# Autodesk Inventor assembly: R-wing
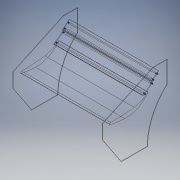
[picture p0: Inventor's stored thumbnail of the model, 180x180]
Saved by Autodesk Inventor 2018.1 (Build 221171000, 171)
## iProperties
Created: 2017-11-02
Part Number: R-wing
Material: 一般
Document SubType Name: Assembly
Designer: kuwano
Author: kuwano
## Documents named in this file (7)
- D:\ku_sk\ドキュメント\Inventor\AeroCAD2018\CAD\Inventor\Aero Parts\R-wing\type6\R-wing.iam
- D:\ku_sk\ドキュメント\Inventor\AeroCAD2018\CAD\Inventor\Aero Parts\R-wing\type6\parts\element_r_1.ipt
- D:\ku_sk\ドキュメント\Inventor\AeroCAD2018\CAD\Inventor\Aero Parts\R-wing\type6\parts\element_r_2.ipt
- D:\ku_sk\ドキュメント\Inventor\AeroCAD2018\CAD\Inventor\Aero Parts\R-wing\type6\parts\end_plate.ipt
- D:\ku_sk\ドキュメント\Inventor\AeroCAD2018\CAD\Inventor\Aero Parts\R-wing\type6\parts\end_plate_MIR.ipt
- D:\ku_sk\ドキュメント\Inventor\AeroCAD2018\CAD\Inventor\Aero Parts\R-wing\type6\parts\cover_re.ipt
- D:\ku_sk\ドキュメント\Inventor\AeroCAD2018\CAD\Inventor\Aero Parts\R-wing\type6\parts\element_clip.ipt
## Components (13 placed, 6 different names)
1. element_r_1:1 — フラッシュ:1, メイト:1, メイト:2, メイト:6, メイト:8, メイト:12, メイト:16, メイト:22, メイト:24, メイト:28, メイト:30
2. element_r_2:1 — フラッシュ:2, メイト:3, メイト:5, メイト:11, メイト:15, メイト:19, メイト:21, メイト:25, メイト:27
3. end_plate:1 — フラッシュ:3, フラッシュ:4, メイト:2, フラッシュ:6, メイト:13, メイト:14, メイト:17, メイト:18, メイト:26, メイト:29
4. end_plate_MIR:1 — フラッシュ:3, フラッシュ:4, メイト:1, メイト:4, メイト:7, メイト:9, メイト:10, メイト:20, メイト:23
5. cover_re:1 — フラッシュ:5
6. element_clip:1 — メイト:3, メイト:4, メイト:5, メイト:10
7. element_clip:2 — メイト:6, メイト:7, メイト:8, メイト:9
8. element_clip:3 — メイト:11, メイト:14, メイト:15, メイト:18
9. element_clip:4 — メイト:12, メイト:13, メイト:16, メイト:17
10. element_clip:5 — メイト:19, メイト:20, メイト:21
11. element_clip:6 — メイト:22, メイト:23, メイト:24
12. element_clip:7 — メイト:25, メイト:26, メイト:27
13. element_clip:8 — メイト:28, メイト:29, メイト:30
## Relationships (36: Mate 30, Flush 6)
- フラッシュ:1 [Flush]: element_r_1:1
- フラッシュ:2 [Flush]: element_r_2:1
- フラッシュ:3 [Flush]: end_plate:1 ↔ end_plate_MIR:1
- フラッシュ:4 [Flush]: end_plate:1 ↔ end_plate_MIR:1
- メイト:1 [Mate]: element_r_1:1 ↔ end_plate_MIR:1
- メイト:2 [Mate]: element_r_1:1 ↔ end_plate:1
- フラッシュ:5 [Flush]: cover_re:1
- メイト:3 [Mate]: element_r_2:1 ↔ element_clip:1
- メイト:4 [Mate]: end_plate_MIR:1 ↔ element_clip:1
- メイト:5 [Mate]: element_r_2:1 ↔ element_clip:1
- メイト:6 [Mate]: element_r_1:1 ↔ element_clip:2
- メイト:7 [Mate]: end_plate_MIR:1 ↔ element_clip:2
- メイト:8 [Mate]: element_r_1:1 ↔ element_clip:2
- メイト:9 [Mate]: end_plate_MIR:1 ↔ element_clip:2
- メイト:10 [Mate]: end_plate_MIR:1 ↔ element_clip:1
- フラッシュ:6 [Flush]: end_plate:1
- メイト:11 [Mate]: element_r_2:1 ↔ element_clip:3
- メイト:12 [Mate]: element_r_1:1 ↔ element_clip:4
- メイト:13 [Mate]: end_plate:1 ↔ element_clip:4
- メイト:14 [Mate]: end_plate:1 ↔ element_clip:3
- メイト:15 [Mate]: element_r_2:1 ↔ element_clip:3
- メイト:16 [Mate]: element_r_1:1 ↔ element_clip:4
- メイト:17 [Mate]: end_plate:1 ↔ element_clip:4
- メイト:18 [Mate]: end_plate:1 ↔ element_clip:3
- メイト:19 [Mate]: element_r_2:1 ↔ element_clip:5
- メイト:20 [Mate]: end_plate_MIR:1 ↔ element_clip:5
- メイト:21 [Mate]: element_r_2:1 ↔ element_clip:5
- メイト:22 [Mate]: element_r_1:1 ↔ element_clip:6
- メイト:23 [Mate]: end_plate_MIR:1 ↔ element_clip:6
- メイト:24 [Mate]: element_r_1:1 ↔ element_clip:6
- メイト:25 [Mate]: element_r_2:1 ↔ element_clip:7
- メイト:26 [Mate]: end_plate:1 ↔ element_clip:7
- メイト:27 [Mate]: element_r_2:1 ↔ element_clip:7
- メイト:28 [Mate]: element_r_1:1 ↔ element_clip:8
- メイト:29 [Mate]: end_plate:1 ↔ element_clip:8
- メイト:30 [Mate]: element_r_1:1 ↔ element_clip:8
